# Autodesk Inventor assembly: wheel1
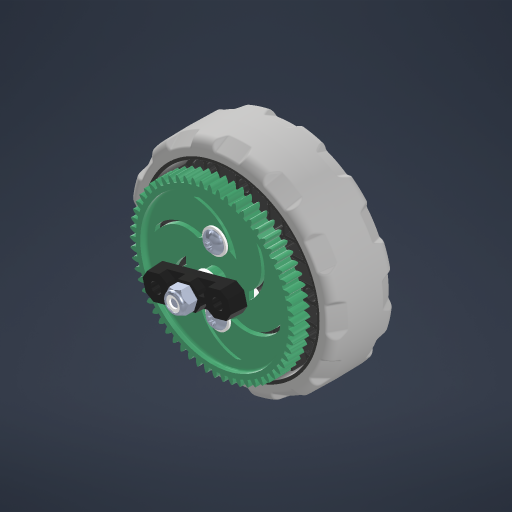
[picture p0: Inventor's stored thumbnail of the model, 512x512]
Saved by Autodesk Inventor 2024 (Build 280153000, 153)
## iProperties
Created: 2023-08-09
Part Number: wheel1
Document SubType Name: Assembly
Designer: macbook
Author: macbook
## Documents named in this file (17)
- \\Mac\Home\Desktop\code\1599V-VRC\Cad\Assembly\v3\tractionwheel.iam
- \\Mac\Home\Desktop\code\1599V-VRC\Cad\Motion\Shaft LS\Bearing Flat.ipt
- \\Mac\Home\Desktop\code\1599V-VRC\Cad\Motion\Spacers\Washer Teflon\TWasher .375 OD x .03125.ipt
- \\Mac\Home\Desktop\code\1599V-VRC\Cad\Structure\Hardware\Nut Nylock.ipt
- \\Mac\Home\Desktop\code\1599V-VRC\Cad\Structure\Hardware\Screw Steel - Star\SScrew Star Smooth 2.500.ipt
- \\Mac\Home\Desktop\code\1599V-VRC\Cad\Motion\Gears\LS 60T Gear.ipt
- \\Mac\Home\Desktop\code\1599V-VRC\Cad\Structure\Hardware\Screw Steel - Star\SScrew Star Threaded 1.250.ipt
- \\Mac\Home\Desktop\code\1599V-VRC\Cad\Motion\Spacers\Spacer Nylon .500 OD\NSpacer White .500 OD x .375.ipt
- \\Mac\Home\Desktop\code\1599V-VRC\Cad\Motion\Spacers\Washer Steel\SWasher .375 OD x .015625.ipt
- \\Mac\Home\Desktop\code\1599V-VRC\Cad\Motion\Spacers\Spacer Nylon .500 OD\NSpacer White .500 OD x .500.ipt
- \\Mac\Home\Desktop\code\1599V-VRC\Cad\Motion\Wheels\Traction Wheel\3.25 Traction AS, Circle.iam
- \\Mac\Home\Desktop\code\1599V-VRC\Cad\Motion\Wheels\Traction Wheel.iam
- \\Mac\Home\Desktop\code\1599V-VRC\Cad\Structure\Hardware\Screw Steel - Star.ipt
- \\Mac\Home\Desktop\code\1599V-VRC\Cad\Motion\Spacers\Spacer Nylon .500 OD.ipt
- \\Mac\Home\Desktop\code\1599V-VRC\Cad\Motion\Spacers\Washer Steel.ipt
- \\Mac\Home\Desktop\code\1599V-VRC\Cad\Motion\Spacers\Washer Teflon.ipt
- \\Mac\Home\Desktop\code\1599V-VRC\Cad\Motion\Spacers\Washer Teflon\TWasher .375 OD x .06250.ipt
## Components (18 placed, 11 different names)
1. Bearing Flat:1
2. Bearing Flat:2 — Insert:30
3. SScrew Star Threaded 1.250:1
4. Nut Nylock:1 — Insert:28
5. Nut Nylock:2 — Insert:25
6. SScrew Star Threaded 1.250:2
7. LS 60T Gear:1 — Insert:27, Insert:29
8. SScrew Star Smooth 2.500:3
9. Nut Nylock:3
10. NSpacer White .500 OD x .500:1 — Insert:22, Insert:26
11. SWasher .375 OD x .015625:1
12. NSpacer White .500 OD x .375:2 — Insert:23, Insert:29
13. TWasher .375 OD x .03125:1
14. TWasher .375 OD x .03125:2
15. NSpacer White .500 OD x .375:3 — Insert:24
16. 3.25 Traction AS, Circle:1 [sub-assembly] — Insert:22, Insert:23, Insert:24, Insert:25, Insert:28
17. TWasher .375 OD x .06250:3 — Insert:27
18. TWasher .375 OD x .06250:4 — Insert:26, Insert:30
## Relationships (19: Insert 19)
- [Insert] (44.45 mm): Bearing Flat:1 ↔ Bearing Flat:2
- [Insert] (44.45 mm): Bearing Flat:1 ↔ Bearing Flat:2
- [Insert] (1.5875 mm): Bearing Flat:2 ↔ SScrew Star Smooth 2.500:3
- [Insert]: Bearing Flat:1 ↔ Nut Nylock:3
- [Insert]: SWasher .375 OD x .015625:1 ↔ NSpacer White .500 OD x .375:2
- [Insert]: SScrew Star Threaded 1.250:1 ↔ TWasher .375 OD x .03125:1
- [Insert]: LS 60T Gear:1 ↔ TWasher .375 OD x .03125:1
- [Insert]: SScrew Star Threaded 1.250:2 ↔ TWasher .375 OD x .03125:2
- [Insert]: LS 60T Gear:1 ↔ TWasher .375 OD x .03125:2
- [Insert]: LS 60T Gear:1 ↔ NSpacer White .500 OD x .375:3
- Insert:22: NSpacer White .500 OD x .500:1 ↔ 3.25 Traction AS, Circle:1
- Insert:23: NSpacer White .500 OD x .375:2 ↔ 3.25 Traction AS, Circle:1
- Insert:24: NSpacer White .500 OD x .375:3 ↔ 3.25 Traction AS, Circle:1
- Insert:25: Nut Nylock:2 ↔ 3.25 Traction AS, Circle:1
- Insert:26: NSpacer White .500 OD x .500:1 ↔ TWasher .375 OD x .06250:4
- Insert:27: LS 60T Gear:1 ↔ TWasher .375 OD x .06250:3
- Insert:28: Nut Nylock:1 ↔ 3.25 Traction AS, Circle:1
- Insert:29: LS 60T Gear:1 ↔ NSpacer White .500 OD x .375:2
- Insert:30: Bearing Flat:2 ↔ TWasher .375 OD x .06250:4
